# Autodesk Inventor assembly: Bras
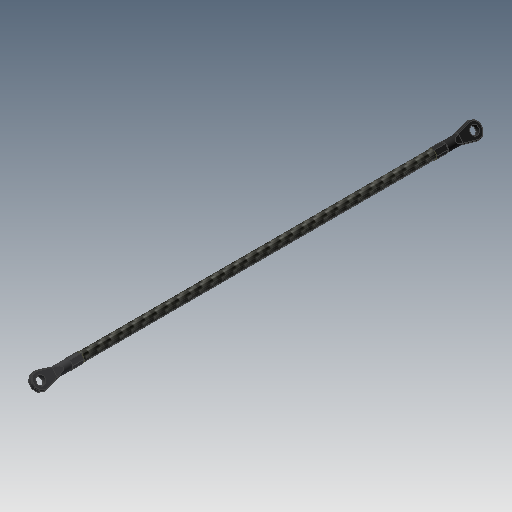
[picture p0: Inventor's stored thumbnail of the model, 512x512]
Saved by Autodesk Inventor 2017 (Build 210142000, 142)
## iProperties
Company: FABLAB Frenchmakers
Part Number: Bras
Material: Générique
Document SubType Name: Assembly
Designer: FABLAB Frenchmakers
Mass: 5.82514 g
Surface Area: 72.7032 cm^2
Volume: 5.57067 cm^3
Density: 1.04568 g/cm^3
Project: 1420 Vauban 3D XL
Catalog Web Link: http://frenchmakers.com/
Stock Number: 1420-10-00
## Documents named in this file (3)
- W:\Professionnel\Conception FABLAB\1420-Vauban 3D XL\1420-10 Bras\1420-10-00 Bras.iam
- W:\Professionnel\Conception FABLAB\1420-Vauban 3D XL\1420-10 Bras\1420-10-01 Bras.ipt
- W:\Professionnel\Conception FABLAB\1420-Vauban 3D XL\1420-10 Bras\1420-10-02 Support rotule.ipt
## Components (3 placed, 2 different names)
1. 1420-10-01 Bras:1 — Affleurement:1, Affleurement:2, Affleurement:3, Placage:1, Placage:2, Placage:3, Placage:4
2. 1420-10-02 Support rotule:1 — Placage:1, Placage:2
3. 1420-10-02 Support rotule:2 — Placage:3, Placage:4
## Relationships (7: Mate 4, Flush 3)
- Affleurement:1 [Flush]: 1420-10-01 Bras:1
- Affleurement:2 [Flush]: 1420-10-01 Bras:1
- Affleurement:3 [Flush]: 1420-10-01 Bras:1
- Placage:1 [Mate]: 1420-10-01 Bras:1 ↔ 1420-10-02 Support rotule:1
- Placage:2 [Mate]: 1420-10-01 Bras:1 ↔ 1420-10-02 Support rotule:1
- Placage:3 [Mate]: 1420-10-01 Bras:1 ↔ 1420-10-02 Support rotule:2
- Placage:4 [Mate]: 1420-10-01 Bras:1 ↔ 1420-10-02 Support rotule:2
